# Autodesk Inventor assembly: 스위치및케이스내부구성도
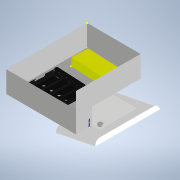
[picture p0: Inventor's stored thumbnail of the model, 180x180]
Saved by Autodesk Inventor 2022 (Build 260153000, 153)
## iProperties
Created: 2022-10-28
Part Number: 스위치및케이스내부구성도
Document SubType Name: Assembly
Designer: Won Hee
Author: Won Hee
## Documents named in this file (7)
- C:\Users\Won Hee\Documents\스위치및케이스내부구성도.iam
- C:\Users\Won Hee\Desktop\sg90-servomotor-1.snapshot.24 - (2)\SG90_Model_B\SG90_Model_B.ipt
- C:\Users\Won Hee\Desktop\sg90-servomotor-1.snapshot.24 - (2)\SG90_Arm_01\SG90_Arm_01 v6.ipt
- C:\Users\Won Hee\Desktop\battery-holder-aasize-1-5v-4-1.snapshot.3\Battery Holder.ipt
- C:\Users\Won Hee\Documents\전체케이스.ipt
- C:\Users\Won Hee\Downloads\스위치.ipt
- C:\Users\Won Hee\Documents\esp32.ipt
## Components (6 placed, 6 different names)
1. SG90_Model_B:1 — 삽입:1, 플러쉬:2
2. SG90_Arm_01 v6:1 — 삽입:1
3. Battery Holder:1 — 플러쉬:1
4. 전체케이스:1 — 메이트:1, 메이트:2, 플러쉬:1, 플러쉬:2, 플러쉬:3
5. 스위치:1 — 메이트:1, 메이트:2
6. esp32:1 — 플러쉬:3
## Relationships (6: Flush 3, Mate 2, Insert 1)
- 삽입:1 [Insert]: SG90_Model_B:1 ↔ SG90_Arm_01 v6:1
- 메이트:1 [Mate]: 전체케이스:1 ↔ 스위치:1
- 메이트:2 [Mate]: 전체케이스:1 ↔ 스위치:1
- 플러쉬:1 [Flush]: Battery Holder:1 ↔ 전체케이스:1
- 플러쉬:2 [Flush]: SG90_Model_B:1 ↔ 전체케이스:1
- 플러쉬:3 [Flush]: 전체케이스:1 ↔ esp32:1
